# Autodesk Inventor assembly: ASY 080 barrel
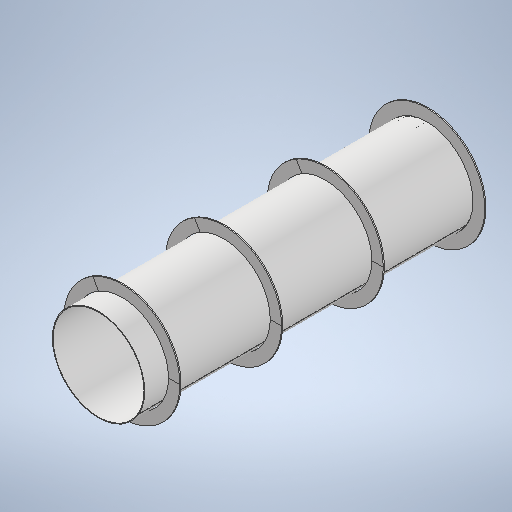
[picture p0: Inventor's stored thumbnail of the model, 512x512]
Saved by Autodesk Inventor 2025 (Build 290162010, 162A)
## iProperties
Created: 2024-08-04
Part Number: ASY 080 barrel
Document SubType Name: Assembly
Designer: pokla
Author: pokla
## Documents named in this file (8)
- C:\Users\DELL\YandexDisk-badmisterfox\домашниий пк\Inventor\BSH_Beshkino_bio_tank\ASY 080 barrel.iam
- C:\Users\DELL\YandexDisk-badmisterfox\домашниий пк\Inventor\BSH_Beshkino_bio_tank\BSH 081 barrel bottom.ipt
- C:\Users\DELL\YandexDisk-badmisterfox\домашниий пк\Inventor\BSH_Beshkino_bio_tank\BSH 082 barrel wall.ipt
- C:\Users\DELL\YandexDisk-badmisterfox\домашниий пк\Inventor\BSH_Beshkino_bio_tank\BSH 083 barrel amplifier.ipt
- C:\Users\DELL\YandexDisk-badmisterfox\домашниий пк\Inventor\BSH_Beshkino_bio_tank\BSH 083 amplifier bottom.ipt
- C:\Users\DELL\YandexDisk-badmisterfox\домашниий пк\Inventor\BSH_Beshkino_bio_tank\BSH 084 amplifier bottom.ipt
- C:\Users\DELL\YandexDisk-badmisterfox\домашниий пк\Inventor\BSH_Beshkino_bio_tank\BSH 085 amplifier bottom.ipt
- C:\Users\DELL\YandexDisk-badmisterfox\домашниий пк\Inventor\BSH_Beshkino_bio_tank\BSH 086 amplifier bottom.ipt
## Components (17 placed, 7 different names)
1. BSH 081 barrel bottom:1
2. BSH 082 barrel wall:1
3. BSH 083 amplifier bottom:1
4. BSH 084 amplifier bottom:1
5. BSH 085 amplifier bottom:1
6. BSH 085 amplifier bottom:2
7. BSH 086 amplifier bottom:1
8. BSH 086 amplifier bottom:2
9. BSH 083 barrel amplifier:1
10. BSH 083 barrel amplifier:2
11. BSH 083 barrel amplifier:3
12. BSH 083 barrel amplifier:4
13. BSH 083 barrel amplifier:5
14. BSH 083 barrel amplifier:6
15. BSH 083 barrel amplifier:7
16. BSH 083 barrel amplifier:8
17. BSH 083 barrel amplifier:9
## Component patterns: (3 elements, first: BSH 083 barrel amplifier:1 + BSH 083 barrel amplifier:2 + BSH 083 barrel amplifier:3)
## Relationships (12: WeldJoint 8, Mate 3, RevoluteJoint 1)
- [RevoluteJoint]: BSH 081 barrel bottom:1 ↔ BSH 082 barrel wall:1
- [WeldJoint]: BSH 083 barrel amplifier:1 ↔ BSH 083 barrel amplifier:2
- [WeldJoint]: BSH 083 barrel amplifier:1 ↔ BSH 083 barrel amplifier:3
- [WeldJoint] (-205 mm): BSH 082 barrel wall:1 ↔ BSH 083 barrel amplifier:2
- [WeldJoint]: BSH 083 amplifier bottom:1 ↔ BSH 084 amplifier bottom:1
- [WeldJoint]: BSH 084 amplifier bottom:1 ↔ BSH 085 amplifier bottom:1
- [WeldJoint]: BSH 084 amplifier bottom:1 ↔ BSH 085 amplifier bottom:2
- [WeldJoint]: BSH 083 amplifier bottom:1 ↔ BSH 086 amplifier bottom:1
- [WeldJoint]: BSH 083 amplifier bottom:1 ↔ BSH 086 amplifier bottom:2
- [Mate]: BSH 081 barrel bottom:1 ↔ BSH 083 amplifier bottom:1
- [Mate]: BSH 081 barrel bottom:1 ↔ BSH 083 amplifier bottom:1
- [Mate]: BSH 081 barrel bottom:1 ↔ BSH 083 amplifier bottom:1
